# Autodesk Inventor assembly: robot7
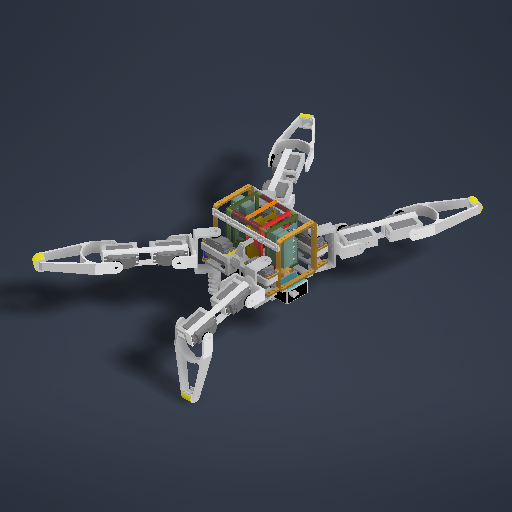
[picture p0: Inventor's stored thumbnail of the model, 512x512]
Saved by Autodesk Inventor 2026.1 (Build 301233000, 233)
## iProperties
Created: 2026-05-07
Part Number: robot7
Document SubType Name: Assembly
Designer: emanuel
Author: emanuel
## Documents named in this file (30)
- C:\Users\emanuel\UnFolder\SpiderRobo\3dmodel\robot7.iam
- C:\Users\emanuel\UnFolder\SpiderRobo\3dmodel\servo_driver.ipt
- C:\Users\emanuel\UnFolder\SpiderRobo\3dmodel\servo_driver_support.ipt
- C:\Users\emanuel\UnFolder\SpiderRobo\3dmodel\small_pillar.ipt
- C:\Users\emanuel\UnFolder\SpiderRobo\3dmodel\wago_support.ipt
- C:\Users\emanuel\UnFolder\SpiderRobo\3dmodel\wago_support_support.ipt
- C:\Users\emanuel\UnFolder\SpiderRobo\3dmodel\individual_servodriver_support.ipt
- C:\Users\emanuel\UnFolder\SpiderRobo\3dmodel\pillar.ipt
- C:\Users\emanuel\UnFolder\SpiderRobo\3dmodel\RP5_support.ipt
- C:\Users\emanuel\UnFolder\SpiderRobo\3dmodel\robot_7_chassis.ipt
- C:\Users\emanuel\UnFolder\SpiderRobo\3dmodel\mg996r.ipt
- C:\Users\emanuel\UnFolder\SpiderRobo\3dmodel\servo_disc.ipt
- C:\Users\emanuel\UnFolder\SpiderRobo\3dmodel\smart_calf.ipt
- C:\Users\emanuel\UnFolder\SpiderRobo\3dmodel\back_servo_support.ipt
- C:\Users\emanuel\UnFolder\SpiderRobo\3dmodel\C2.ipt
- C:\Users\emanuel\UnFolder\SpiderRobo\3dmodel\femur.ipt
- C:\Users\emanuel\UnFolder\SpiderRobo\3dmodel\servo_support_4.ipt
- C:\Users\emanuel\UnFolder\SpiderRobo\3dmodel\C1.ipt
- C:\Users\emanuel\UnFolder\SpiderRobo\3dmodel\shoe.ipt
- C:\Users\emanuel\UnFolder\SpiderRobo\3dmodel\link1.ipt
- C:\Users\emanuel\UnFolder\SpiderRobo\3dmodel\link2.ipt
- C:\Users\emanuel\UnFolder\SpiderRobo\3dmodel\small_pillar2.ipt
- C:\Users\emanuel\UnFolder\SpiderRobo\3dmodel\back_servo_support2.ipt
- C:\Users\emanuel\UnFolder\SpiderRobo\3dmodel\structural_ring1.ipt
- C:\Users\emanuel\UnFolder\SpiderRobo\3dmodel\structural_bar1.ipt
- C:\Users\emanuel\UnFolder\SpiderRobo\3dmodel\pillar1.ipt
- C:\Users\emanuel\UnFolder\SpiderRobo\3dmodel\piulita.ipt
- C:\Users\emanuel\UnFolder\SpiderRobo\3dmodel\battery1.ipt
- C:\Users\emanuel\UnFolder\SpiderRobo\3dmodel\battery_holder_2.ipt
- C:\Users\emanuel\UnFolder\SpiderRobo\3dmodel\leg.ipt
## Components (120 placed, 29 different names)
1. servo_driver:1 — Mate:44, Mate:45, Mate:46
2. servo_driver_support:1 — Mate:32, Mate:33, Mate:34
3. small_pillar:1 — Mate:1, Mate:2, Mate:20, Mate:21
4. wago_support:1 — Mate:38, Mate:39, Mate:40
5. wago_support_support:1 — Mate:35, Mate:36, Mate:37, Mate:38, Mate:39, Mate:40
6. individual_servodriver_support:1 — Mate:1, Mate:2, Mate:3, Mate:4, Mate:5, Mate:6, Mate:7, Mate:8, Mate:19, Mate:22, Mate:25, Mate:28, Mate:44, Mate:45, Mate:46
7. pillar:1 — Mate:26, Mate:27, Mate:28, Mate:29, Mate:30
8. RP5_support:1 — Mate:29, Mate:30, Mate:31, Mate:32, Mate:33, Mate:34, Mate:41, Mate:42, Mate:43, Mate:257, Mate:261, Mate:262, Mate:263
9. small_pillar:2 — Mate:7, Mate:8, Mate:23, Mate:24
10. small_pillar:3 — Mate:5, Mate:6, Mate:26, Mate:27
11. small_pillar:4 — Mate:3, Mate:4, Mate:17, Mate:18
12. small_pillar:5 — Mate:41
13. individual_servodriver_support:2 — Mate:42, Mate:43, Mate:47, Mate:48, Mate:49
14. small_pillar:6
15. small_pillar:7
16. small_pillar:8
17. pillar:2 — Mate:23, Mate:24, Mate:25
18. pillar:3 — Mate:17, Mate:18, Mate:19, Mate:35, Mate:37
19. pillar:4 — Mate:20, Mate:21, Mate:22, Mate:31, Mate:36
20. servo_driver:2 — Mate:47, Mate:48, Mate:49
21. robot_7_chassis:1 — Mate:228, Mate:229, Mate:231, Mate:232, Mate:234, Mate:235, Mate:237, Mate:238, Mate:247, Mate:248, Mate:249, Mate:254, Mate:255, Mate:256, Mate:258, Mate:259, Mate:260, Mate:262, Mate:289, Mate:291, Mate:293, Mate:294, Mate:295, Mate:296, Mate:297, Mate:298, Mate:299, Mate:300, Mate:301, Mate:302, Mate:303, Mate:304, Mate:313, Mate:314, Mate:315, Mate:324, Mate:325, Mate:326, Mate:328, Mate:329, Mate:330, Mate:331, Mate:332, Mate:335
22. mg996r:1 — Mate:228, Mate:229, Mate:306
23. servo_disc:1
24. smart_calf:1
25. servo_disc:2
26. back_servo_support:1
27. C2:1
28. femur:1
29. mg996r:2
30. servo_disc:3
31. mg996r:3
32. back_servo_support:2
33. servo_support_4:1
34. servo_support_4:2
35. servo_support_4:3
36. servo_support_4:4
37. C1:1
38. shoe:1
39. mg996r:4 — Mate:237, Mate:238, Mate:316, Mate:333, Mate:334
40. servo_disc:4
41. smart_calf:2
42. servo_disc:5
43. back_servo_support:3
44. C2:2
45. femur:2
46. mg996r:5
47. servo_disc:6
48. mg996r:6
49. back_servo_support:4
50. servo_support_4:5
51. servo_support_4:6
52. servo_support_4:7
53. servo_support_4:8
54. C1:2 — Mate:358, Mate:359
55. shoe:2
56. mg996r:7 — Mate:231, Mate:232, Mate:317
57. servo_disc:7
58. smart_calf:3
59. servo_disc:8
60. back_servo_support:5
61. C2:3
62. femur:3
63. mg996r:8
64. servo_disc:9
65. mg996r:9
66. back_servo_support:6
67. servo_support_4:9
68. servo_support_4:10
69. servo_support_4:11
70. servo_support_4:12
71. C1:3
72. shoe:3
73. mg996r:10 — Mate:234, Mate:235, Mate:305, Mate:336, Mate:337
74. servo_disc:10
75. smart_calf:4
76. servo_disc:11
77. back_servo_support:7
78. C2:4
79. femur:4
80. mg996r:11
81. servo_disc:12
82. mg996r:12
83. back_servo_support:8
84. servo_support_4:13
85. servo_support_4:14
86. servo_support_4:15
87. servo_support_4:16
88. C1:4
89. shoe:4
90. servo_support_4:17 — Mate:247, Mate:248, Mate:249
91. link1:1 — Mate:254, Mate:255, Mate:256, Mate:257, Mate:264
92. link2:1 — Mate:258, Mate:259, Mate:260, Mate:261
93. small_pillar2:1 — Mate:263, Mate:264
94. servo_support_4:19
95. servo_support_4:21 — Mate:291
96. servo_support_4:23 — Mate:289, Mate:293, Mate:294, Mate:295
97. link1:2 — Mate:296, Mate:297, Mate:298
98. link2:2 — Mate:299, Mate:300, Mate:301
99. structural_bar1:1
100. structural_bar1:3
101. structural_ring1:1 — Mate:302, Mate:303, Mate:304, Mate:305, Mate:306, Mate:307, Mate:308, Mate:309, Mate:310, Mate:311, Mate:312, Mate:338, Mate:339, Mate:340, Mate:341, Mate:342, Mate:343, Mate:344, Mate:345, Mate:346, Mate:347, Flush:1
102. structural_ring1:2 — Mate:313, Mate:314, Mate:315, Mate:316, Mate:317, Mate:318, Mate:319, Mate:320, Mate:321, Mate:322, Mate:323, Mate:348, Mate:349
103. back_servo_support2:4 — Mate:310, Mate:311, Mate:312
104. back_servo_support2:5 — Mate:307, Mate:308, Mate:309
105. back_servo_support2:7 — Mate:318, Mate:319, Mate:320
106. back_servo_support2:8 — Mate:321, Mate:322, Mate:323, Mate:327
107. pillar1:1 — Mate:324, Mate:325
108. pillar1:2 — Mate:326, Mate:327
109. pillar1:3 — Mate:330, Mate:331
110. pillar1:4 — Mate:328, Mate:329
111. piulita:1 — Mate:332, Mate:333, Mate:334
112. piulita:2 — Mate:335, Mate:336, Mate:337
113. battery1:1 — Mate:356, Mate:357, Flush:1
114. structural_bar1:4 — Mate:338, Mate:339, Mate:340, Mate:350
115. structural_bar1:5 — Mate:341, Mate:342, Mate:343, Mate:351, Mate:352, Mate:353, Mate:354, Mate:355
116. structural_bar1:6 — Mate:344, Mate:345, Mate:346
117. structural_bar1:7 — Mate:347, Mate:348, Mate:349
118. battery_holder_2:1 — Mate:350, Mate:351, Mate:352, Mate:357
119. battery_holder_2:2 — Mate:353, Mate:354, Mate:355, Mate:356
120. leg:1 — Mate:358, Mate:359
## Relationships (317: Mate 316, Flush 1)
- Mate:1: small_pillar:1 ↔ individual_servodriver_support:1
- Mate:2: small_pillar:1 ↔ individual_servodriver_support:1
- Mate:3: individual_servodriver_support:1 ↔ small_pillar:4
- Mate:4: individual_servodriver_support:1 ↔ small_pillar:4
- Mate:5: individual_servodriver_support:1 ↔ small_pillar:3
- Mate:6: individual_servodriver_support:1 ↔ small_pillar:3
- Mate:7: individual_servodriver_support:1 ↔ small_pillar:2
- Mate:8: individual_servodriver_support:1 ↔ small_pillar:2
- [Mate]: small_pillar:5 ↔ individual_servodriver_support:2
- [Mate]: small_pillar:5 ↔ individual_servodriver_support:2
- [Mate]: individual_servodriver_support:2 ↔ small_pillar:8
- [Mate]: individual_servodriver_support:2 ↔ small_pillar:8
- [Mate]: individual_servodriver_support:2 ↔ small_pillar:7
- [Mate]: individual_servodriver_support:2 ↔ small_pillar:7
- [Mate]: individual_servodriver_support:2 ↔ small_pillar:6
- [Mate]: individual_servodriver_support:2 ↔ small_pillar:6
- Mate:17: small_pillar:4 ↔ pillar:3
- Mate:18: small_pillar:4 ↔ pillar:3
- Mate:19: individual_servodriver_support:1 ↔ pillar:3
- Mate:20: small_pillar:1 ↔ pillar:4
- Mate:21: small_pillar:1 ↔ pillar:4
- Mate:22: individual_servodriver_support:1 ↔ pillar:4
- Mate:23: small_pillar:2 ↔ pillar:2
- Mate:24: small_pillar:2 ↔ pillar:2
- Mate:25: individual_servodriver_support:1 ↔ pillar:2
- Mate:26: pillar:1 ↔ small_pillar:3
- Mate:27: pillar:1 ↔ small_pillar:3
- Mate:28: individual_servodriver_support:1 ↔ pillar:1
- Mate:29: pillar:1 ↔ RP5_support:1
- Mate:30: pillar:1 ↔ RP5_support:1
- Mate:31: RP5_support:1 ↔ pillar:4
- Mate:32: servo_driver_support:1 ↔ RP5_support:1
- Mate:33: servo_driver_support:1 ↔ RP5_support:1
- Mate:34: servo_driver_support:1 ↔ RP5_support:1
- Mate:35: wago_support_support:1 ↔ pillar:3
- Mate:36: wago_support_support:1 ↔ pillar:4
- Mate:37: wago_support_support:1 ↔ pillar:3
- Mate:38: wago_support:1 ↔ wago_support_support:1
- Mate:39: wago_support:1 ↔ wago_support_support:1
- Mate:40: wago_support:1 ↔ wago_support_support:1
- Mate:41: RP5_support:1 ↔ small_pillar:5
- Mate:42: RP5_support:1 ↔ individual_servodriver_support:2
- Mate:43: RP5_support:1 ↔ individual_servodriver_support:2
- Mate:44: servo_driver:1 ↔ individual_servodriver_support:1
- Mate:45: servo_driver:1 ↔ individual_servodriver_support:1
- Mate:46: servo_driver:1 ↔ individual_servodriver_support:1
- Mate:47: individual_servodriver_support:2 ↔ servo_driver:2
- Mate:48: individual_servodriver_support:2 ↔ servo_driver:2
- Mate:49: individual_servodriver_support:2 ↔ servo_driver:2
- [Mate]: mg996r:1 ↔ servo_disc:1
- [Mate]: mg996r:1 ↔ servo_disc:1
- [Mate]: servo_disc:2 ↔ mg996r:2
- [Mate]: servo_disc:2 ↔ mg996r:2
- [Mate]: servo_disc:3 ↔ mg996r:3
- [Mate]: servo_disc:3 ↔ mg996r:3
- [Mate]: femur:1 ↔ mg996r:3
- [Mate]: femur:1 ↔ mg996r:3
- [Mate]: femur:1 ↔ mg996r:3
- [Mate]: femur:1 ↔ mg996r:2
- [Mate]: femur:1 ↔ mg996r:2
- [Mate]: femur:1 ↔ mg996r:2
- [Mate]: C2:1 ↔ servo_disc:3
- [Mate]: C2:1 ↔ mg996r:3
- [Mate]: femur:1 ↔ servo_support_4:1
- [Mate]: femur:1 ↔ servo_support_4:4
- [Mate]: femur:1 ↔ servo_support_4:2
- [Mate]: femur:1 ↔ servo_support_4:3
- [Mate]: femur:1 ↔ servo_support_4:1
- [Mate]: mg996r:2 ↔ servo_support_4:4
- [Mate]: back_servo_support:2 ↔ servo_support_4:1
- [Mate]: back_servo_support:2 ↔ servo_support_4:1
- [Mate]: back_servo_support:2 ↔ servo_support_4:1
- [Mate]: back_servo_support:2 ↔ servo_support_4:4
- [Mate]: femur:1 ↔ servo_support_4:1
- [Mate]: femur:1 ↔ servo_support_4:3
- [Mate]: femur:1 ↔ servo_support_4:3
- [Mate]: mg996r:3 ↔ servo_support_4:2
- [Mate]: back_servo_support:1 ↔ servo_support_4:3
- [Mate]: back_servo_support:1 ↔ servo_support_4:3
- [Mate]: back_servo_support:1 ↔ servo_support_4:3
- [Mate]: back_servo_support:1 ↔ servo_support_4:2
- [Mate]: smart_calf:1 ↔ servo_disc:2
- [Mate]: smart_calf:1 ↔ mg996r:2
- [Mate]: C2:1 ↔ C1:1
- [Mate]: C2:1 ↔ C1:1
- [Mate]: C2:1 ↔ C1:1
- [Mate]: C2:1 ↔ C1:1
- [Mate]: C2:1 ↔ C1:1
- [Mate]: servo_disc:1 ↔ C1:1
- [Mate]: mg996r:1 ↔ C1:1
- [Mate]: smart_calf:1 ↔ shoe:1
- [Mate]: smart_calf:1 ↔ shoe:1
- [Mate]: smart_calf:1 ↔ shoe:1
- [Mate]: mg996r:4 ↔ servo_disc:4
- [Mate]: mg996r:4 ↔ servo_disc:4
- [Mate]: servo_disc:5 ↔ mg996r:5
- [Mate]: servo_disc:5 ↔ mg996r:5
- [Mate]: servo_disc:6 ↔ mg996r:6
- [Mate]: servo_disc:6 ↔ mg996r:6
- [Mate]: femur:2 ↔ mg996r:6
- [Mate]: femur:2 ↔ mg996r:6
- [Mate]: femur:2 ↔ mg996r:6
- [Mate]: femur:2 ↔ mg996r:5
- [Mate]: femur:2 ↔ mg996r:5
- [Mate]: femur:2 ↔ mg996r:5
- [Mate]: C2:2 ↔ servo_disc:6
- [Mate]: C2:2 ↔ mg996r:6
- [Mate]: femur:2 ↔ servo_support_4:5
- [Mate]: femur:2 ↔ servo_support_4:8
- [Mate]: femur:2 ↔ servo_support_4:6
- [Mate]: femur:2 ↔ servo_support_4:7
- [Mate]: femur:2 ↔ servo_support_4:5
- [Mate]: mg996r:5 ↔ servo_support_4:8
- [Mate]: back_servo_support:4 ↔ servo_support_4:5
- [Mate]: back_servo_support:4 ↔ servo_support_4:5
- [Mate]: back_servo_support:4 ↔ servo_support_4:5
- [Mate]: back_servo_support:4 ↔ servo_support_4:8
- [Mate]: femur:2 ↔ servo_support_4:5
- [Mate]: femur:2 ↔ servo_support_4:7
- [Mate]: femur:2 ↔ servo_support_4:7
- [Mate]: mg996r:6 ↔ servo_support_4:6
- [Mate]: back_servo_support:3 ↔ servo_support_4:7
- [Mate]: back_servo_support:3 ↔ servo_support_4:7
- [Mate]: back_servo_support:3 ↔ servo_support_4:7
- [Mate]: back_servo_support:3 ↔ servo_support_4:6
- [Mate]: smart_calf:2 ↔ servo_disc:5
- [Mate]: smart_calf:2 ↔ mg996r:5
- [Mate]: C2:2 ↔ C1:2
- [Mate]: C2:2 ↔ C1:2
- [Mate]: C2:2 ↔ C1:2
- [Mate]: C2:2 ↔ C1:2
- [Mate]: C2:2 ↔ C1:2
- [Mate]: servo_disc:4 ↔ C1:2
- [Mate]: mg996r:4 ↔ C1:2
- [Mate]: smart_calf:2 ↔ shoe:2
- [Mate]: smart_calf:2 ↔ shoe:2
- [Mate]: smart_calf:2 ↔ shoe:2
- [Mate]: mg996r:7 ↔ servo_disc:7
- [Mate]: mg996r:7 ↔ servo_disc:7
- [Mate]: servo_disc:8 ↔ mg996r:8
- [Mate]: servo_disc:8 ↔ mg996r:8
- [Mate]: servo_disc:9 ↔ mg996r:9
- [Mate]: servo_disc:9 ↔ mg996r:9
- [Mate]: femur:3 ↔ mg996r:9
- [Mate]: femur:3 ↔ mg996r:9
- [Mate]: femur:3 ↔ mg996r:9
- [Mate]: femur:3 ↔ mg996r:8
- [Mate]: femur:3 ↔ mg996r:8
- [Mate]: femur:3 ↔ mg996r:8
- [Mate]: C2:3 ↔ servo_disc:9
- [Mate]: C2:3 ↔ mg996r:9
- [Mate]: femur:3 ↔ servo_support_4:9
- [Mate]: femur:3 ↔ servo_support_4:12
- [Mate]: femur:3 ↔ servo_support_4:10
- [Mate]: femur:3 ↔ servo_support_4:11
- [Mate]: femur:3 ↔ servo_support_4:9
- [Mate]: mg996r:8 ↔ servo_support_4:12
- [Mate]: back_servo_support:6 ↔ servo_support_4:9
- [Mate]: back_servo_support:6 ↔ servo_support_4:9
- [Mate]: back_servo_support:6 ↔ servo_support_4:9
- [Mate]: back_servo_support:6 ↔ servo_support_4:12
- [Mate]: femur:3 ↔ servo_support_4:9
- [Mate]: femur:3 ↔ servo_support_4:11
- [Mate]: femur:3 ↔ servo_support_4:11
- [Mate]: mg996r:9 ↔ servo_support_4:10
- [Mate]: back_servo_support:5 ↔ servo_support_4:11
- [Mate]: back_servo_support:5 ↔ servo_support_4:11
- [Mate]: back_servo_support:5 ↔ servo_support_4:11
- [Mate]: back_servo_support:5 ↔ servo_support_4:10
- [Mate]: smart_calf:3 ↔ servo_disc:8
- [Mate]: smart_calf:3 ↔ mg996r:8
- [Mate]: C2:3 ↔ C1:3
- [Mate]: C2:3 ↔ C1:3
- [Mate]: C2:3 ↔ C1:3
- [Mate]: C2:3 ↔ C1:3
- [Mate]: C2:3 ↔ C1:3
- [Mate]: servo_disc:7 ↔ C1:3
- [Mate]: mg996r:7 ↔ C1:3
- [Mate]: smart_calf:3 ↔ shoe:3
- [Mate]: smart_calf:3 ↔ shoe:3
- [Mate]: smart_calf:3 ↔ shoe:3
- [Mate]: mg996r:10 ↔ servo_disc:10
- [Mate]: mg996r:10 ↔ servo_disc:10
- [Mate]: servo_disc:11 ↔ mg996r:11
- [Mate]: servo_disc:11 ↔ mg996r:11
- [Mate]: servo_disc:12 ↔ mg996r:12
- [Mate]: servo_disc:12 ↔ mg996r:12
- [Mate]: femur:4 ↔ mg996r:12
- [Mate]: femur:4 ↔ mg996r:12
- [Mate]: femur:4 ↔ mg996r:12
- [Mate]: femur:4 ↔ mg996r:11
- [Mate]: femur:4 ↔ mg996r:11
- [Mate]: femur:4 ↔ mg996r:11
- [Mate]: C2:4 ↔ servo_disc:12
- [Mate]: C2:4 ↔ mg996r:12
- [Mate]: femur:4 ↔ servo_support_4:13
- [Mate]: femur:4 ↔ servo_support_4:16
- [Mate]: femur:4 ↔ servo_support_4:14
- [Mate]: femur:4 ↔ servo_support_4:15
- [Mate]: femur:4 ↔ servo_support_4:13
- [Mate]: mg996r:11 ↔ servo_support_4:16
- [Mate]: back_servo_support:8 ↔ servo_support_4:13
- [Mate]: back_servo_support:8 ↔ servo_support_4:13
- [Mate]: back_servo_support:8 ↔ servo_support_4:13
- [Mate]: back_servo_support:8 ↔ servo_support_4:16
- [Mate]: femur:4 ↔ servo_support_4:13
- [Mate]: femur:4 ↔ servo_support_4:15
- [Mate]: femur:4 ↔ servo_support_4:15
- [Mate]: mg996r:12 ↔ servo_support_4:14
- [Mate]: back_servo_support:7 ↔ servo_support_4:15
- [Mate]: back_servo_support:7 ↔ servo_support_4:15
- [Mate]: back_servo_support:7 ↔ servo_support_4:15
- [Mate]: back_servo_support:7 ↔ servo_support_4:14
- [Mate]: smart_calf:4 ↔ servo_disc:11
- [Mate]: smart_calf:4 ↔ mg996r:11
- [Mate]: C2:4 ↔ C1:4
- [Mate]: C2:4 ↔ C1:4
- [Mate]: C2:4 ↔ C1:4
- [Mate]: C2:4 ↔ C1:4
- [Mate]: C2:4 ↔ C1:4
- [Mate]: servo_disc:10 ↔ C1:4
- [Mate]: mg996r:10 ↔ C1:4
- [Mate]: smart_calf:4 ↔ shoe:4
- [Mate]: smart_calf:4 ↔ shoe:4
- [Mate]: smart_calf:4 ↔ shoe:4
- Mate:228: robot_7_chassis:1 ↔ mg996r:1
- Mate:229: robot_7_chassis:1 ↔ mg996r:1
- Mate:231: robot_7_chassis:1 ↔ mg996r:7
- Mate:232: robot_7_chassis:1 ↔ mg996r:7
- Mate:234: robot_7_chassis:1 ↔ mg996r:10
- Mate:235: robot_7_chassis:1 ↔ mg996r:10
- Mate:237: robot_7_chassis:1 ↔ mg996r:4
- Mate:238: robot_7_chassis:1 ↔ mg996r:4
- Mate:247: robot_7_chassis:1 ↔ servo_support_4:17
- Mate:248: robot_7_chassis:1 ↔ servo_support_4:17
- Mate:249: robot_7_chassis:1 ↔ servo_support_4:17
- Mate:254: robot_7_chassis:1 ↔ link1:1
- Mate:255: robot_7_chassis:1 ↔ link1:1
- Mate:256: robot_7_chassis:1 ↔ link1:1
- Mate:257: RP5_support:1 ↔ link1:1
- Mate:258: robot_7_chassis:1 ↔ link2:1
- Mate:259: robot_7_chassis:1 ↔ link2:1
- Mate:260: robot_7_chassis:1 ↔ link2:1
- Mate:261: RP5_support:1 ↔ link2:1
- Mate:262 (5.65 mm): RP5_support:1 ↔ robot_7_chassis:1
- Mate:263: RP5_support:1 ↔ small_pillar2:1
- Mate:264: link1:1 ↔ small_pillar2:1
- Mate:289: robot_7_chassis:1 ↔ servo_support_4:23
- Mate:291: robot_7_chassis:1 ↔ servo_support_4:21
- Mate:293: robot_7_chassis:1 ↔ servo_support_4:23
- Mate:294: robot_7_chassis:1 ↔ servo_support_4:23
- Mate:295: robot_7_chassis:1 ↔ servo_support_4:23
- Mate:296: robot_7_chassis:1 ↔ link1:2
- Mate:297: robot_7_chassis:1 ↔ link1:2
- Mate:298: robot_7_chassis:1 ↔ link1:2
- Mate:299: robot_7_chassis:1 ↔ link2:2
- Mate:300: robot_7_chassis:1 ↔ link2:2
- Mate:301: robot_7_chassis:1 ↔ link2:2
- Mate:302: robot_7_chassis:1 ↔ structural_ring1:1
- Mate:303: robot_7_chassis:1 ↔ structural_ring1:1
- Mate:304: robot_7_chassis:1 ↔ structural_ring1:1
- Mate:305: mg996r:10 ↔ structural_ring1:1
- Mate:306: mg996r:1 ↔ structural_ring1:1
- Mate:307: structural_ring1:1 ↔ back_servo_support2:5
- Mate:308: structural_ring1:1 ↔ back_servo_support2:5
- Mate:309: structural_ring1:1 ↔ back_servo_support2:5
- Mate:310: structural_ring1:1 ↔ back_servo_support2:4
- Mate:311: structural_ring1:1 ↔ back_servo_support2:4
- Mate:312: structural_ring1:1 ↔ back_servo_support2:4
- Mate:313: robot_7_chassis:1 ↔ structural_ring1:2
- Mate:314: robot_7_chassis:1 ↔ structural_ring1:2
- Mate:315: robot_7_chassis:1 ↔ structural_ring1:2
- Mate:316: mg996r:4 ↔ structural_ring1:2
- Mate:317: mg996r:7 ↔ structural_ring1:2
- Mate:318: structural_ring1:2 ↔ back_servo_support2:7
- Mate:319: structural_ring1:2 ↔ back_servo_support2:7
- Mate:320: structural_ring1:2 ↔ back_servo_support2:7
- Mate:321: structural_ring1:2 ↔ back_servo_support2:8
- Mate:322: structural_ring1:2 ↔ back_servo_support2:8
- Mate:323: structural_ring1:2 ↔ back_servo_support2:8
- Mate:324: robot_7_chassis:1 ↔ pillar1:1
- Mate:325: robot_7_chassis:1 ↔ pillar1:1
- Mate:326: robot_7_chassis:1 ↔ pillar1:2
- Mate:327: back_servo_support2:8 ↔ pillar1:2
- Mate:328: robot_7_chassis:1 ↔ pillar1:4
- Mate:329: robot_7_chassis:1 ↔ pillar1:4
- Mate:330: robot_7_chassis:1 ↔ pillar1:3
- Mate:331: robot_7_chassis:1 ↔ pillar1:3
- Mate:332: robot_7_chassis:1 ↔ piulita:1
- Mate:333: mg996r:4 ↔ piulita:1
- Mate:334: mg996r:4 ↔ piulita:1
- Mate:335: robot_7_chassis:1 ↔ piulita:2
- Mate:336: mg996r:10 ↔ piulita:2
- Mate:337: mg996r:10 ↔ piulita:2
- Mate:338: structural_ring1:1 ↔ structural_bar1:4
- Mate:339: structural_ring1:1 ↔ structural_bar1:4
- Mate:340: structural_ring1:1 ↔ structural_bar1:4
- Mate:341: structural_ring1:1 ↔ structural_bar1:5
- Mate:342: structural_ring1:1 ↔ structural_bar1:5
- Mate:343: structural_ring1:1 ↔ structural_bar1:5
- Mate:344: structural_ring1:1 ↔ structural_bar1:6
- Mate:345: structural_ring1:1 ↔ structural_bar1:6
- Mate:346: structural_ring1:1 ↔ structural_bar1:6
- Mate:347: structural_ring1:1 ↔ structural_bar1:7
- Mate:348: structural_ring1:2 ↔ structural_bar1:7
- Mate:349: structural_ring1:2 ↔ structural_bar1:7
- Mate:350: structural_bar1:4 ↔ battery_holder_2:1
- Mate:351: structural_bar1:5 ↔ battery_holder_2:1
- Mate:352: structural_bar1:5 ↔ battery_holder_2:1
- Mate:353: structural_bar1:5 ↔ battery_holder_2:2
- Mate:354: structural_bar1:5 ↔ battery_holder_2:2
- Mate:355: structural_bar1:5 ↔ battery_holder_2:2
- Mate:356: battery1:1 ↔ battery_holder_2:2
- Mate:357: battery1:1 ↔ battery_holder_2:1
- Flush:1: structural_ring1:1 ↔ battery1:1
- Mate:358: C1:2 ↔ leg:1
- Mate:359: C1:2 ↔ leg:1
## Named parameters: d8_d0 = 0 mm, d9_d1 = 0 mm, d10_d2 = 0 mm, d11_d3 = 0 mm, d12_d4 = 0 mm, d13_d5 = 0 mm, d14_d6 = 0 mm, d15_d7 = 0 mm, d305_d226 = 0 mm, d306_d227 = 0 mm, d307_d228 = 0 mm, d308_d229 = 0 mm, d309_d155 = 0 mm, d310_d156 = 0 mm, d311_d125_d101 = 0 mm, d312_d126_d102 = 0 mm, d313_d127_d103 = 0 mm, d314_d128_d104 = 0 mm, d315_d129_d105 = 0 mm, d316_d130_d106 = 0 mm, d317_d131_d107 = 0 mm, d318_d132_d108 = 0 mm, d319_d133_d109 = 0 mm, d320_d134_d110 = 0 mm, d321_d135_d111 = 0 mm, d322_d136_d112 = 0 mm, d323_d137_d113 = 0 mm, d324_d138_d114 = 0 mm, d325_d139_d115 = 0 mm, d326_d140_d116 = 0 mm, d327_d141_d117 = 0 mm, d328_d142_d118 = 0 mm, d329_d143_d119 = 0 mm, d330_d144_d120 = 0 mm, d331_d145_d121 = 0 mm, d332_d146_d122 = 0 mm, d333_d147_d123 = 0 mm, d334_d148_d124 = 0 mm, d335_d149_d95 = 0 mm, d336_d150_d96 = 0 mm, d337_d151_d97_d95 = 0 mm, d338_d152_d98_d96 = 0 mm, d339_d153_d99 = 0 mm, d340_d154_d100 = 0 mm, d341_d230 = 0 mm, d63_d37 = 0 mm, d64_d38 = 0 mm, d96_d487 = 0 mm, d97_d488 = 0 mm, d98_d489 = 0 mm, d99_d305_d226 = 0 mm, d100_d306_d227 = 0 mm, d101_d307_d228 = 0 mm, d102_d308_d229 = 0 mm, d103_d309_d155 = 0 mm, d104_d310_d156 = 0 mm, d105_d311_d125_d101 = 0 mm, d106_d312_d126_d102 = 0 mm, d107_d313_d127_d103 = 0 mm, d108_d314_d128_d104 = 0 mm, d109_d315_d129_d105 = 0 mm, d110_d316_d130_d106 = 0 mm, d111_d317_d131_d107 = 0 mm, d112_d318_d132_d108 = 0 mm, d113_d319_d133_d109 = 0 mm, d114_d320_d134_d110 = 0 mm, d115_d321_d135_d111 = 0 mm, d116_d322_d136_d112 = 0 mm, d117_d323_d137_d113 = 0 mm, d118_d324_d138_d114 = 0 mm, d119_d325_d139_d115 = 0 mm, d120_d326_d140_d116 = 0 mm, d121_d327_d141_d117 = 0 mm, d122_d328_d142_d118 = 0 mm, d123_d329_d143_d119 = 0 mm, d124_d330_d144_d120 = 0 mm, d125_d331_d145_d121 = 0 mm, d126_d332_d146_d122 = 0 mm, d127_d333_d147_d123 = 0 mm, d128_d334_d148_d124 = 0 mm, d129_d335_d149_d95 = 0 mm, d130_d336_d150_d96 = 0 mm, d131_d337_d151_d97_d95 = 0 mm, d132_d338_d152_d98_d96 = 0 mm, d133_d339_d153_d99 = 0 mm, d134_d340_d154_d100 = 0 mm, d135_d341_d230 = 0 mm, d136_d342 = 0 mm, d137_d343 = 0 mm, d138_d63_d37 = 0 mm, d139_d64_d38 = 0 mm, d140_d487 = 0 mm, d141_d488 = 0 mm, d142_d489 = 0 mm, d143_d305_d226 = 0 mm, d144_d306_d227 = 0 mm, d145_d307_d228 = 0 mm, d146_d308_d229 = 0 mm, d147_d309_d155 = 0 mm, d148_d310_d156 = 0 mm, d149_d311_d125_d101 = 0 mm, d150_d312_d126_d102 = 0 mm, d151_d313_d127_d103 = 0 mm, d152_d314_d128_d104 = 0 mm, d153_d315_d129_d105 = 0 mm, d154_d316_d130_d106 = 0 mm, d155_d317_d131_d107 = 0 mm, d156_d318_d132_d108 = 0 mm, d157_d319_d133_d109 = 0 mm, d158_d320_d134_d110 = 0 mm, d159_d321_d135_d111 = 0 mm, d160_d322_d136_d112 = 0 mm, d161_d323_d137_d113 = 0 mm, d162_d324_d138_d114 = 0 mm, d163_d325_d139_d115 = 0 mm, d164_d326_d140_d116 = 0 mm, d165_d327_d141_d117 = 0 mm, d166_d328_d142_d118 = 0 mm, d167_d329_d143_d119 = 0 mm, d168_d330_d144_d120 = 0 mm, d169_d331_d145_d121 = 0 mm, d170_d332_d146_d122 = 0 mm, d171_d333_d147_d123 = 0 mm, d172_d334_d148_d124 = 0 mm, d173_d335_d149_d95 = 0 mm, d174_d336_d150_d96 = 0 mm, d175_d337_d151_d97_d95 = 0 mm, d176_d338_d152_d98_d96 = 0 mm, d177_d339_d153_d99 = 0 mm, d178_d340_d154_d100 = 0 mm, d179_d341_d230 = 0 mm, d180_d342 = 0 mm, d181_d343 = 0 mm, d182_d63_d37 = 0 mm, d183_d64_d38 = 0 mm, d184_d487 = 0 mm, d185_d488 = 0 mm, d186_d489 = 0 mm, d187_d305_d226 = 0 mm, d188_d306_d227 = 0 mm, d189_d307_d228 = 0 mm, d190_d308_d229 = 0 mm, d191_d309_d155 = 0 mm, d192_d310_d156 = 0 mm, d193_d311_d125_d101 = 0 mm, d194_d312_d126_d102 = 0 mm, d195_d313_d127_d103 = 0 mm, d196_d314_d128_d104 = 0 mm, d197_d315_d129_d105 = 0 mm, d198_d316_d130_d106 = 0 mm, d199_d317_d131_d107 = 0 mm, d200_d318_d132_d108 = 0 mm, d201_d319_d133_d109 = 0 mm, d202_d320_d134_d110 = 0 mm, d203_d321_d135_d111 = 0 mm, d204_d322_d136_d112 = 0 mm, d205_d323_d137_d113 = 0 mm, d206_d324_d138_d114 = 0 mm, d207_d325_d139_d115 = 0 mm, d208_d326_d140_d116 = 0 mm, d209_d327_d141_d117 = 0 mm, d210_d328_d142_d118 = 0 mm, d211_d329_d143_d119 = 0 mm, d212_d330_d144_d120 = 0 mm, d213_d331_d145_d121 = 0 mm, d214_d332_d146_d122 = 0 mm, d215_d333_d147_d123 = 0 mm, d216_d334_d148_d124 = 0 mm, d217_d335_d149_d95 = 0 mm, d218_d336_d150_d96 = 0 mm, d219_d337_d151_d97_d95 = 0 mm, d220_d338_d152_d98_d96 = 0 mm, d221_d339_d153_d99 = 0 mm, d222_d340_d154_d100 = 0 mm, d223_d341_d230 = 0 mm, d224_d342 = 0 mm, d225_d343 = 0 mm, d226_d63_d37 = 0 mm, d227_d64_d38 = 0 mm
